# Autodesk Inventor assembly: frame
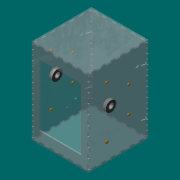
[picture p0: Inventor's stored thumbnail of the model, 180x180]
Saved by Autodesk Inventor 2016 (Build 200138000, 138)
## iProperties
Created: 2015-10-05
Part Number: frame
Document SubType Name: Assembly
Designer: Sawaiz
Author: Sawaiz
## Documents named in this file (6)
- C:\Users\sawaiz\oneDrive\projects\splitFlapDisplay\frame\frame.iam
- C:\Users\sawaiz\oneDrive\projects\splitFlapDisplay\frame\front.ipt
- C:\Users\sawaiz\oneDrive\projects\splitFlapDisplay\frame\back.ipt
- C:\Users\sawaiz\oneDrive\projects\splitFlapDisplay\frame\topBottomPanel.ipt
- C:\Users\sawaiz\oneDrive\projects\splitFlapDisplay\frame\leftSide.iam
- C:\Users\sawaiz\oneDrive\projects\splitFlapDisplay\frame\rightSide.iam
## Components (6 placed, 5 different names)
1. front:1 — Flush:2, Mate:2, Flush:4, Mate:4, Flush:5, Flush:6, Flush:8, Flush:10, Flush:11
2. topBottomPanel:1 — Flush:2, Mate:2, Flush:7, Flush:9, Flush:12, Flush:13, Flush:14, Flush:15
3. topBottomPanel:2 — Flush:4, Mate:4, Flush:5
4. leftSide:1 [sub-assembly] — Flush:6, Flush:7, Flush:8
5. rightSide:1 [sub-assembly] — Flush:9, Flush:10, Flush:11, Flush:15
6. back:1 — Flush:12, Flush:13, Flush:14
## Relationships (15: Flush 13, Mate 2)
- Flush:2: front:1 ↔ topBottomPanel:1
- Mate:2: front:1 ↔ topBottomPanel:1
- Flush:4: front:1 ↔ topBottomPanel:2
- Mate:4: front:1 ↔ topBottomPanel:2
- Flush:5: front:1 ↔ topBottomPanel:2
- Flush:6: front:1 ↔ leftSide:1
- Flush:7: topBottomPanel:1 ↔ leftSide:1
- Flush:8: front:1 ↔ leftSide:1
- Flush:9: topBottomPanel:1 ↔ rightSide:1
- Flush:10: front:1 ↔ rightSide:1
- Flush:11: front:1 ↔ rightSide:1
- Flush:12: topBottomPanel:1 ↔ back:1
- Flush:13: topBottomPanel:1 ↔ back:1
- Flush:14: topBottomPanel:1 ↔ back:1
- Flush:15: topBottomPanel:1 ↔ rightSide:1
